# Autodesk Inventor assembly: Chuck with BBM Staging Plate
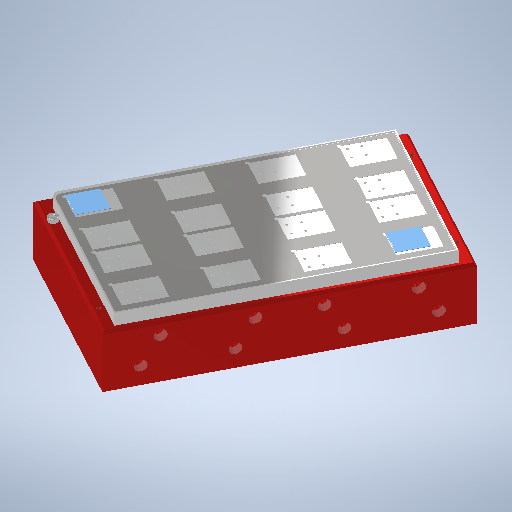
[picture p0: Inventor's stored thumbnail of the model, 512x512]
Saved by Autodesk Inventor 2025 (Build 290162000, 162)
## iProperties
Created: 2021-11-09
Part Number: Chuck with BBM Staging Plate
Document SubType Name: Assembly
Designer: Caleb
Author: Caleb
## Documents named in this file (3)
- C:\Users\cfang\Desktop\nebraska-silicon-lab\Hardware\ETL\Module Assembly\Chuck - 16-pocket V1\Chuck with BBM Staging Plate.iam
- C:\Users\cfang\Desktop\nebraska-silicon-lab\Hardware\ETL\Module Assembly\Chuck - 16-pocket V1\Chuck - 16-pocket.iam
- C:\Users\cfang\Desktop\nebraska-silicon-lab\Hardware\ETL\Module Assembly\BBM Staging Plate - V2\BBM Staging Plate Assembly - V2.iam
## Components (2 placed, 2 different names)
1. Chuck - 16-pocket:1 [sub-assembly] — Mate:1, Angle:1, Tangent:1, Tangent:2
2. BBM Staging Plate Assembly - V2:1 [sub-assembly] — Mate:1, Angle:1, Tangent:1, Tangent:2
## Relationships (4: Tangent 2, Mate 1, Angle 1)
- Mate:1: Chuck - 16-pocket:1 ↔ BBM Staging Plate Assembly - V2:1
- Angle:1 (0 deg): Chuck - 16-pocket:1 ↔ BBM Staging Plate Assembly - V2:1
- Tangent:1: Chuck - 16-pocket:1 ↔ BBM Staging Plate Assembly - V2:1
- Tangent:2: Chuck - 16-pocket:1 ↔ BBM Staging Plate Assembly - V2:1
